# Autodesk Inventor assembly: 2415-C01
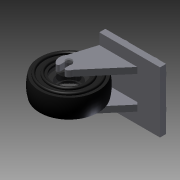
[picture p0: Inventor's stored thumbnail of the model, 180x180]
Saved by Autodesk Inventor 2011 SP1 (Build 150282100, 282)
## iProperties
Created: 2011-09-28
Part Number: 2415-C01
Cost Center: 0 kg
Document SubType Name: Assembly
Designer: PMe
Authority: 0 mm^3
Stock Number: =<Filenr>_<Document number>
Company: Allseas Engineering BV
Subject: =<Title><TITLE 1_2> <TITLE 2_2>
Author: PMe
Act. Code: DW000
SaveDate: 2011-06-29
SaveTime: 11:35
FileName: Standard
TotalMass: 0 kg
TotalVolume: 0 mm^3
## Documents named in this file (4)
- C:\Documents and Settings\pme\My Documents\fun folder\LEGO-VLIEGTUIG\2415-C01.iam
- C:\Documents and Settings\pme\My Documents\fun folder\LEGO-VLIEGTUIG\2415.ipt
- C:\Documents and Settings\pme\My Documents\fun folder\LEGO-VLIEGTUIG\3139.ipt
- C:\Documents and Settings\pme\My Documents\fun folder\LEGO-VLIEGTUIG\3464.ipt
## Components (3 placed, 3 different names)
1. 2415:1 — Insert:1
2. 3139:1 — Insert:2
3. 3464:1 — Insert:1, Insert:2
## Relationships (2: Insert 2)
- Insert:1: 2415:1 ↔ 3464:1
- Insert:2: 3139:1 ↔ 3464:1
